# Autodesk Inventor assembly: s-assy-cover-right
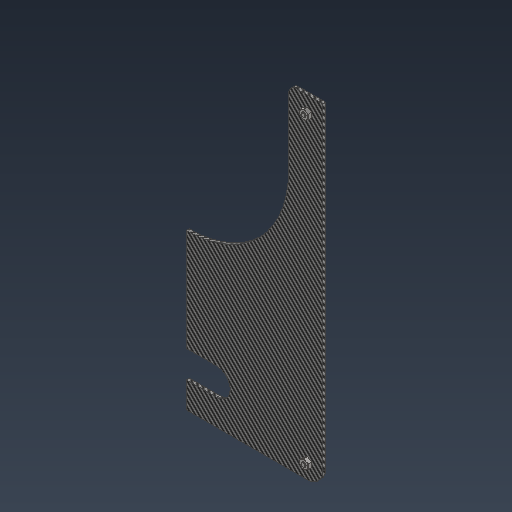
[picture p0: Inventor's stored thumbnail of the model, 512x512]
Saved by Autodesk Inventor 2021 (Build 250183000, 183)
## iProperties
Created: 2021-08-05
Part Number: s-assy-cover-right
Document SubType Name: Assembly
Designer: yuta0
Author: yuta0
## Documents named in this file (4)
- C:\Users\yuta0\Documents\GitHub\catchrobo_hardware\catchrobo_robot\s-assy-cover-right.iam
- C:\Users\yuta0\Documents\GitHub\catchrobo_hardware\catchrobo_robot\carbon_plate5.ipt
- C:\Users\yuta0\Documents\GitHub\catchrobo_hardware\catchrobo_robot\CB3-5.ipt
- C:\Users\yuta0\Documents\GitHub\catchrobo_hardware\catchrobo_robot\LBNR3.ipt
## Components (5 placed, 3 different names)
1. carbon_plate5:1 — メイト:1, メイト:2, メイト:4
2. CB3-5:1 — メイト:1, メイト:2, メイト:3
3. LBNR3:1 — メイト:3, メイト:4
4. CB3-5:2
5. LBNR3:2
## Component patterns: (2 elements, first: CB3-5:1 + LBNR3:1)
## Relationships (4: Mate 4)
- メイト:1 [Mate]: carbon_plate5:1 ↔ CB3-5:1
- メイト:2 [Mate]: carbon_plate5:1 ↔ CB3-5:1
- メイト:3 [Mate]: CB3-5:1 ↔ LBNR3:1
- メイト:4 [Mate]: carbon_plate5:1 ↔ LBNR3:1
